# Autodesk Inventor assembly: 1111_Magnet Brick SubAssembly_V1
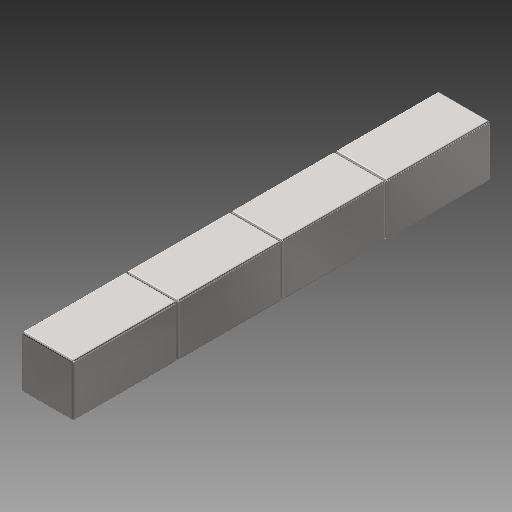
[picture p0: Inventor's stored thumbnail of the model, 512x512]
Saved by Autodesk Inventor 2020 (Build 240168000, 168)
## iProperties
Created: 2019-10-13
Part Number: 1111_Magnet Brick SubAssembly_V1
Document SubType Name: Assembly
Designer: RFLab
Author: RFLab
## Documents named in this file (2)
- C:\Users\RFLab\Dropbox\MPI Group Folder\fMPI (Rodent)\Small Bore Imager_Open Source Files\Inventor Files\1xxx_Rotating Gantry\11xx_Magnet Assembly\111x_Permanent Magnets\1111_Magnet Brick SubAssembly_V1.iam
- C:\Users\RFLab\Dropbox\MPI Group Folder\fMPI (Rodent)\Small Bore Imager_Open Source Files\Inventor Files\1xxx_Rotating Gantry\11xx_Magnet Assembly\111x_Permanent Magnets\1111A_Individual NdFeB Block_V1.ipt
## Components (4 placed, 1 different names)
1. 1111A_Individual NdFeB Block_V1:1 — Flush:1, Flush:2, Mate:1, Mate:2, Mate:3, Mate:4, Mate:6, Flush:5, Flush:6
2. 1111A_Individual NdFeB Block_V1:2 — Flush:1, Flush:2, Mate:1
3. 1111A_Individual NdFeB Block_V1:3
4. 1111A_Individual NdFeB Block_V1:4 — Mate:6, Flush:5, Flush:6
## Relationships (12: Flush 6, Mate 6)
- Flush:1: 1111A_Individual NdFeB Block_V1:1 ↔ 1111A_Individual NdFeB Block_V1:2
- Flush:2: 1111A_Individual NdFeB Block_V1:1 ↔ 1111A_Individual NdFeB Block_V1:2
- Mate:1: 1111A_Individual NdFeB Block_V1:1 ↔ 1111A_Individual NdFeB Block_V1:2
- Mate:2: 1111A_Individual NdFeB Block_V1:1
- Mate:3: 1111A_Individual NdFeB Block_V1:1
- Mate:4: 1111A_Individual NdFeB Block_V1:1
- [Flush]: 1111A_Individual NdFeB Block_V1:3 ↔ 1111A_Individual NdFeB Block_V1:4
- [Flush]: 1111A_Individual NdFeB Block_V1:3 ↔ 1111A_Individual NdFeB Block_V1:4
- [Mate]: 1111A_Individual NdFeB Block_V1:3 ↔ 1111A_Individual NdFeB Block_V1:4
- Mate:6: 1111A_Individual NdFeB Block_V1:1 ↔ 1111A_Individual NdFeB Block_V1:4
- Flush:5: 1111A_Individual NdFeB Block_V1:1 ↔ 1111A_Individual NdFeB Block_V1:4
- Flush:6: 1111A_Individual NdFeB Block_V1:1 ↔ 1111A_Individual NdFeB Block_V1:4
## Named parameters: d6_d2 = 0 mm, d7_d0 = 0 mm, d8_d1 = 0 mm
